# Autodesk Inventor assembly: 6P Sprocket
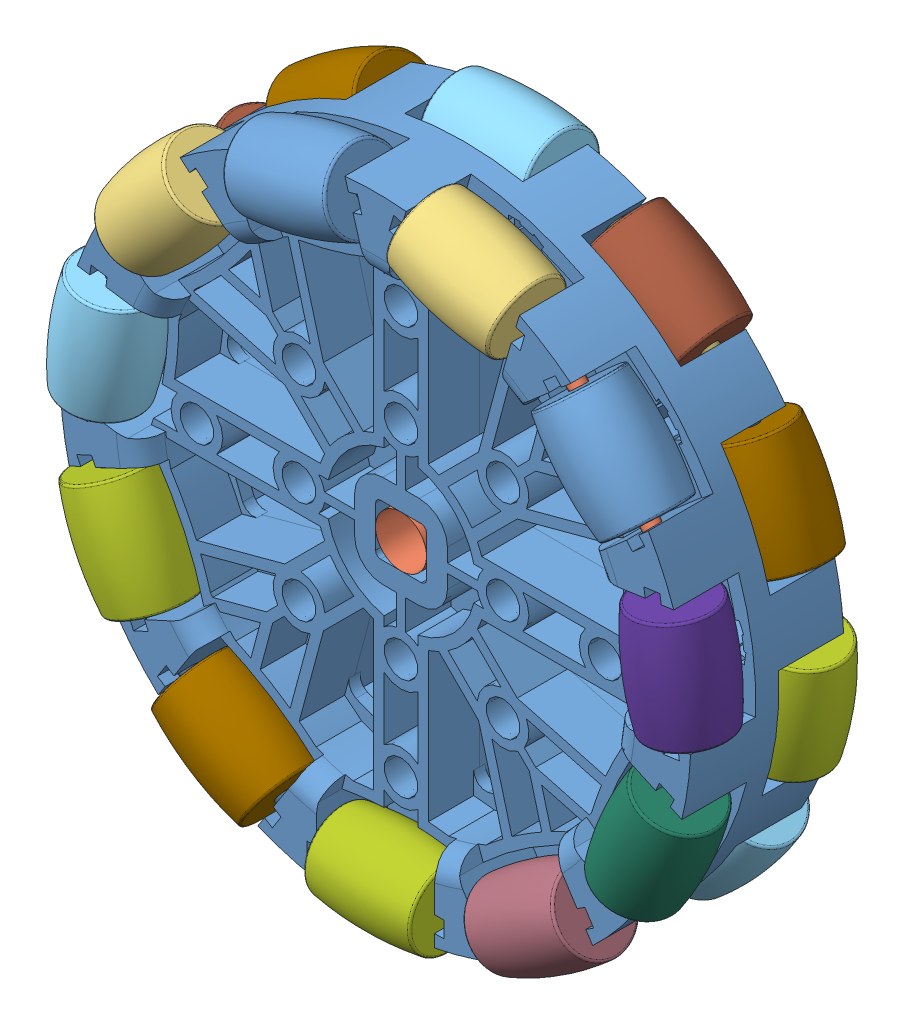
[picture p0: shaded view drawn from the shape stored in the file]
Saved by Autodesk Inventor 2023 (Build 270158000, 158)
## iProperties
Created: 2022-08-02
Part Number: 6P Sprocket
Document SubType Name: Assembly
Designer: ylu12
Author: ylu12
## Documents named in this file (3)
- D:\Documents\Inventor\VEX\Library Backup\Library 1.4\Motion\Wheels\Omni Wheel\3.25 Omni AS, No Insert.iam
- D:\Documents\Inventor\VEX\Library Backup\Library 1.4\Motion\Wheels\Reference Files\3.25 Omni Antistatic.ipt
- D:\Documents\Inventor\VEX\Library Backup\Library 1.4\Motion\Wheels\Omni Wheel.iam
## Components (1 placed, 1 different names)
1. 3.25 Omni Antistatic
## Relationships (3: Mate 2, Flush 1)
- [Flush]: 3.25 Omni Antistatic
- [Mate]: 3.25 Omni Antistatic
- [Mate]: 3.25 Omni Antistatic
